# Autodesk Inventor assembly: Mounting Plate Assemly
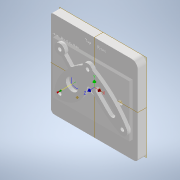
[picture p0: Inventor's stored thumbnail of the model, 180x180]
Saved by Autodesk Inventor 2021 (Build 250183000, 183)
## iProperties
Created: 2021-05-20
Part Number: Mounting Plate Assemly
Document SubType Name: Assembly
Designer: maza168
Author: maza168
## Documents named in this file (4)
- \\unifiles.uoa.auckland.ac.nz\myhome\Documents\334\Project B\NC Files Submission 2\Mounting Plate Assemly.iam
- \\unifiles.uoa.auckland.ac.nz\myhome\Documents\334\NC Files Submission\Template.ipt
- \\unifiles.uoa.auckland.ac.nz\myhome\Documents\334\NC Files Submission\y3_design_mounting_plate_2018.ipt
- \\unifiles.uoa.auckland.ac.nz\myhome\Documents\334\Project B\NC Files Submission 2\Final Bracket Design.ipt
## Components (3 placed, 3 different names)
1. Template:1 — Rigid:1
2. y3_design_mounting_plate_2018:1 — Rigid:1, Mate:3, Mate:4, Mate:5, Mate:6, Mate:7, Mate:8
3. Final Bracket Design:1 — Mate:6, Mate:7, Mate:8
## Relationships (7: Mate 6, WeldJoint 1)
- Rigid:1 [WeldJoint]: Template:1 ↔ y3_design_mounting_plate_2018:1
- Mate:3: y3_design_mounting_plate_2018:1
- Mate:4: y3_design_mounting_plate_2018:1
- Mate:5: y3_design_mounting_plate_2018:1
- Mate:6: y3_design_mounting_plate_2018:1 ↔ Final Bracket Design:1
- Mate:7: y3_design_mounting_plate_2018:1 ↔ Final Bracket Design:1
- Mate:8: y3_design_mounting_plate_2018:1 ↔ Final Bracket Design:1
